# Autodesk Inventor assembly: LegUpperBackLinkUnit_MIR
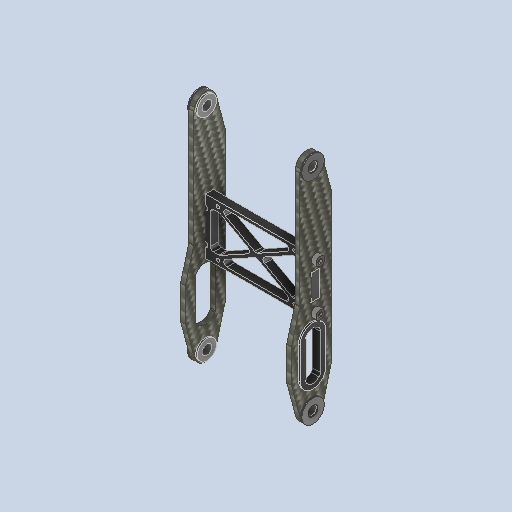
[picture p0: Inventor's stored thumbnail of the model, 512x512]
Saved by Autodesk Inventor 2024.2 (Build 282272000, 272)
## iProperties
Created: 2024-01-06
Part Number: LegUpperBackLinkUnit_MIR
Document SubType Name: Assembly
Designer: Masato Kubotera
Mass: 40.5776 g
Surface Area: 239.681 cm^2
Volume: 21.0227 cm^3
Density: 1.93018 g/cm^3
Author: Masato Kubotera
## Documents named in this file (8)
- C:\Users\masato\OneDrive - Chiba Institute of Technology\CIT Brains\RoboCup2024\Mechanic\SUSTAINA-OP2-DEV\NativeFiles\Boby\LowerLimb\Legs\Links\LegUpperBackLinkUnit_MIR.iam
- C:\Users\masato\OneDrive - Chiba Institute of Technology\CIT Brains\RoboCup2024\Mechanic\SUSTAINA-OP2-DEV\NativeFiles\Boby\LowerLimb\Legs\Links\LegLinkBraceFrame.ipt
- C:\Users\masato\OneDrive - Chiba Institute of Technology\CIT Brains\RoboCup2024\Mechanic\SUSTAINA-OP2-DEV\NativeFiles\Boby\LowerLimb\Legs\Links\LegBackLinkFrame.ipt
- C:\Users\masato\OneDrive - Chiba Institute of Technology\CIT Brains\RoboCup2024\Mechanic\SUSTAINA-OP2-DEV\NativeFiles\Boby\COTS\Screws\CapScrew\UC-0308.ipt
- C:\Users\masato\OneDrive - Chiba Institute of Technology\CIT Brains\RoboCup2024\Mechanic\SUSTAINA-OP2-DEV\NativeFiles\Boby\COTS\Bushes\GFM-0608-04.ipt
- C:\Users\masato\OneDrive - Chiba Institute of Technology\CIT Brains\RoboCup2024\Mechanic\SUSTAINA-OP2-DEV\NativeFiles\Boby\CommonDesignedComponents\SliderProtectionFrame.ipt
- C:\Users\masato\OneDrive - Chiba Institute of Technology\CIT Brains\RoboCup2024\Mechanic\SUSTAINA-OP2-DEV\NativeFiles\Boby\COTS\Washers\Resin\TT-0614-05.ipt
- C:\Users\masato\OneDrive - Chiba Institute of Technology\CIT Brains\RoboCup2024\Mechanic\SUSTAINA-OP2-DEV\NativeFiles\Boby\COTS\Washers\Metal\UUW-0614-05H.ipt
## Components (20 placed, 7 different names)
1. LegBackLinkFrame:1 — Insert:1, Insert:2, Insert:5, Insert:6, Insert:13, Insert:14, Insert:17, Insert:18, Insert:21, Insert:22
2. LegBackLinkFrame:2 — Insert:3, Insert:4, Insert:7, Insert:8, Insert:15, Insert:16, Insert:19, Insert:20
3. LegLinkBraceFrame:1 — Insert:1, Insert:2, Insert:3, Insert:4, Flush:1, Angle:1
4. SliderProtectionFrame:1 — Insert:21, Insert:22
5. GFM-0608-04:1 — Insert:17
6. GFM-0608-04:2 — Insert:18, Mate:1
7. GFM-0608-04:3 — Insert:19
8. GFM-0608-04:4 — Insert:20
9. UC-0308:1 — Insert:13
10. UC-0308:2 — Insert:14
11. UC-0308:3 — Insert:15
12. UC-0308:4 — Insert:16
13. TT-0614-05:4 — Insert:5, Insert:9
14. TT-0614-05:1 — Insert:6, Insert:10
15. TT-0614-05:3 — Insert:7, Insert:11
16. TT-0614-05:2 — Insert:8, Insert:12
17. UUW-0614-05H:1 — Insert:9
18. UUW-0614-05H:2 — Insert:10
19. UUW-0614-05H:3 — Insert:11
20. UUW-0614-05H:4 — Insert:12
## Relationships (25: Insert 22, Mate 1, Flush 1, Angle 1)
- Insert:1: LegBackLinkFrame:1 ↔ LegLinkBraceFrame:1
- Insert:2: LegBackLinkFrame:1 ↔ LegLinkBraceFrame:1
- Insert:3: LegBackLinkFrame:2 ↔ LegLinkBraceFrame:1
- Insert:4: LegBackLinkFrame:2 ↔ LegLinkBraceFrame:1
- Mate:1: GFM-0608-04:2
- Flush:1: LegLinkBraceFrame:1
- Angle:1 (0 deg): LegLinkBraceFrame:1
- Insert:5: LegBackLinkFrame:1 ↔ TT-0614-05:4
- Insert:6: LegBackLinkFrame:1 ↔ TT-0614-05:1
- Insert:7: LegBackLinkFrame:2 ↔ TT-0614-05:3
- Insert:8: LegBackLinkFrame:2 ↔ TT-0614-05:2
- Insert:9: TT-0614-05:4 ↔ UUW-0614-05H:1
- Insert:10: TT-0614-05:1 ↔ UUW-0614-05H:2
- Insert:11: TT-0614-05:3 ↔ UUW-0614-05H:3
- Insert:12: TT-0614-05:2 ↔ UUW-0614-05H:4
- Insert:13: LegBackLinkFrame:1 ↔ UC-0308:1
- Insert:14: LegBackLinkFrame:1 ↔ UC-0308:2
- Insert:15: LegBackLinkFrame:2 ↔ UC-0308:3
- Insert:16: LegBackLinkFrame:2 ↔ UC-0308:4
- Insert:17: LegBackLinkFrame:1 ↔ GFM-0608-04:1
- Insert:18: LegBackLinkFrame:1 ↔ GFM-0608-04:2
- Insert:19: LegBackLinkFrame:2 ↔ GFM-0608-04:3
- Insert:20: LegBackLinkFrame:2 ↔ GFM-0608-04:4
- Insert:21: LegBackLinkFrame:1 ↔ SliderProtectionFrame:1
- Insert:22: LegBackLinkFrame:1 ↔ SliderProtectionFrame:1
